# Autodesk Inventor assembly: GFBL85050-250-SET
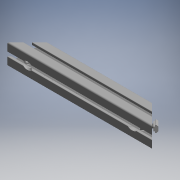
[picture p0: Inventor's stored thumbnail of the model, 180x180]
Saved by Autodesk Inventor 2017.3 (Build 213256000, 256)
## iProperties
Category: PARTsolutions
Company: MISUMI
Part Number: GFBL85050-250-SET
Catalog Web Link: www.cadenas.de
Description: GFBL8-4545,GFBL8-4590,GFBL8-5050,GFBL8-50100-Brackets for Reinforcement - HFS8-45 Series-
Vendor: MISUMI
Document SubType Name: Assembly
Designer: partserver
Manufacturer: MISUMI
Mass: 496.59 g
Surface Area: 1307.48 cm^2
Volume: 496.59 cm^3
Density: 1 g/cm^3
Title: GFBL85050-250-SET
Author: Cadenas PARTsolutions
Comments: Brackets for Reinforcement - HFS8-45 Series-
PSOL_IDENT_0: {$CADENAS_DATA\23d-libs\misumi\metric\38_al_extrusions_blackets\8_45\gfbl8_45_asmtab.prj},233 {VTYP=
PSOL_IDENT_1: 3D},{STYP=ASSTAB},{NB=GFBL85050-250-SET},{LINA=GFBL85050-250-SET},{NN=GFBL8-4545,GFBL8-4590,GFBL8-50
PSOL_IDENT_2: 50,GFBL8-50100},{DATE=08.06.2021 08:26:11},{GEOMDATE=23.05.2017 05:01:27},{VERSION=},{LINEID=30},{WB
PSOL_IDENT_3: VAR=L,ALT1},{WBNUMERIC=L}  {NB=GFBL85050-250-SET},{LINA=GFBL85050-250-SET},{KT=DUMMY},{PN=GFBL85050-
PSOL_IDENT_4: 250-SET},{TYPE=GFBL8},{NO=5050},{L=250},{ALT1=-SET},{PPATH=gfbl8_45/gfbl8_45_asmtpl.prj}
NB: GFBL85050-250-SET
NN: GFBL8-4545,GFBL8-4590,GFBL8-5050,GFBL8-50100
NT: Brackets for Reinforcement - HFS8-45 Series-
NBSYN: $PN.
LINA: GFBL85050-250-SET
CATALOG: Misumi
PN: GFBL85050-250-SET
TYPE: GFBL8
NO: 5050
L: 250
ALT1: SET Applicable Screws and Nuts Set
SUPPLIER: MISUMI
ARTICLENO: GFBL85050-250-SET
BOMINFO: GFBL85050-250-SET
CREATOR: CADENAS GmbH
## Documents named in this file (6)
- e:\temp\worker_65\temp\exporttempdir_10092_110_zDKcX\format_0\GFBL85050-250-SET.iam
- e:\temp\worker_65\temp\exporttempdir_10092_110_zDKcX\format_0\GFBL85050-250-SET_b.ipt
- e:\temp\worker_65\temp\exporttempdir_10092_110_zDKcX\format_0\HCBST8-24_Screw.ipt
- e:\temp\worker_65\temp\exporttempdir_10092_110_zDKcX\format_0\HCBST8_w1.ipt
- e:\temp\worker_65\temp\exporttempdir_10092_110_zDKcX\format_0\HCBST8washer2.ipt
- e:\temp\worker_65\temp\exporttempdir_10092_110_zDKcX\format_0\HNTT8-8.ipt
## Components (9 placed, 5 different names)
1. GFBL85050-250-SET_b:1 — to_bolt21_XY@1 <-> screw_to_body_XY@2, to_bolt21_Z@1 <-> screw_to_body_Z@2, to_bolt21_YZ@1 <-> screw_to_body_YZ@2, to_bolt22_XY@1 <-> screw_to_body_XY@5, to_bolt22_Z@1 <-> screw_to_body_Z@5, to_bolt22_YZ@1 <-> screw_to_body_YZ@5, to_nut21_XY@1 <-> to_bolt_XY@8, to_nut21_Z@1 <-> to_bolt_Z@8, to_nut21_YZ@1 <-> to_bolt_YZ@8, to_nut22_XY@1 <-> to_bolt_XY@9, to_nut22_Z@1 <-> to_bolt_Z@9, to_nut22_YZ@1 <-> to_bolt_YZ@9
2. HCBST8-24_Screw:1 — to_bolt21_XY@1 <-> screw_to_body_XY@2, to_bolt21_Z@1 <-> screw_to_body_Z@2, to_bolt21_YZ@1 <-> screw_to_body_YZ@2, bolt_to_spring_washer_XY@2 <-> spring_washer_to_bolt_XY@3, bolt_to_spring_washer_Z@2 <-> spring_washer_to_bolt_Z@3, bolt_to_spring_washer_YZ@2 <-> spring_washer_to_bolt_YZ@3, bolt_to_plane_washer_XY@2 <-> washer_to_bolt_XY@4, bolt_to_plane_washer_Z@2 <-> washer_to_bolt_Z@4, bolt_to_plane_washer_YZ@2 <-> washer_to_bolt_YZ@4
3. HCBST8_w1:1 — bolt_to_spring_washer_XY@2 <-> spring_washer_to_bolt_XY@3, bolt_to_spring_washer_Z@2 <-> spring_washer_to_bolt_Z@3, bolt_to_spring_washer_YZ@2 <-> spring_washer_to_bolt_YZ@3
4. HCBST8washer2:1 — bolt_to_plane_washer_XY@2 <-> washer_to_bolt_XY@4, bolt_to_plane_washer_Z@2 <-> washer_to_bolt_Z@4, bolt_to_plane_washer_YZ@2 <-> washer_to_bolt_YZ@4
5. HCBST8-24_Screw:2 — to_bolt22_XY@1 <-> screw_to_body_XY@5, to_bolt22_Z@1 <-> screw_to_body_Z@5, to_bolt22_YZ@1 <-> screw_to_body_YZ@5, bolt_to_spring_washer_XY@5 <-> spring_washer_to_bolt_XY@6, bolt_to_spring_washer_Z@5 <-> spring_washer_to_bolt_Z@6, bolt_to_spring_washer_YZ@5 <-> spring_washer_to_bolt_YZ@6, bolt_to_plane_washer_XY@5 <-> washer_to_bolt_XY@7, bolt_to_plane_washer_Z@5 <-> washer_to_bolt_Z@7, bolt_to_plane_washer_YZ@5 <-> washer_to_bolt_YZ@7
6. HCBST8_w1:2 — bolt_to_spring_washer_XY@5 <-> spring_washer_to_bolt_XY@6, bolt_to_spring_washer_Z@5 <-> spring_washer_to_bolt_Z@6, bolt_to_spring_washer_YZ@5 <-> spring_washer_to_bolt_YZ@6
7. HCBST8washer2:2 — bolt_to_plane_washer_XY@5 <-> washer_to_bolt_XY@7, bolt_to_plane_washer_Z@5 <-> washer_to_bolt_Z@7, bolt_to_plane_washer_YZ@5 <-> washer_to_bolt_YZ@7
8. HNTT8-8:1 — to_nut21_XY@1 <-> to_bolt_XY@8, to_nut21_Z@1 <-> to_bolt_Z@8, to_nut21_YZ@1 <-> to_bolt_YZ@8
9. HNTT8-8:2 — to_nut22_XY@1 <-> to_bolt_XY@9, to_nut22_Z@1 <-> to_bolt_Z@9, to_nut22_YZ@1 <-> to_bolt_YZ@9
## Relationships (24: Mate 14, Angle 8, Flush 2)
- to_bolt21_XY@1 <-> screw_to_body_XY@2 [Mate] (4.2 mm): GFBL85050-250-SET_b:1 ↔ HCBST8-24_Screw:1
- to_bolt21_Z@1 <-> screw_to_body_Z@2 [Mate]: GFBL85050-250-SET_b:1 ↔ HCBST8-24_Screw:1
- to_bolt21_YZ@1 <-> screw_to_body_YZ@2 [Angle] (0 deg): GFBL85050-250-SET_b:1 ↔ HCBST8-24_Screw:1
- bolt_to_spring_washer_XY@2 <-> spring_washer_to_bolt_XY@3 [Mate] (-2.8 mm): HCBST8-24_Screw:1 ↔ HCBST8_w1:1
- bolt_to_spring_washer_Z@2 <-> spring_washer_to_bolt_Z@3 [Mate]: HCBST8-24_Screw:1 ↔ HCBST8_w1:1
- bolt_to_spring_washer_YZ@2 <-> spring_washer_to_bolt_YZ@3 [Angle] (0 deg): HCBST8-24_Screw:1 ↔ HCBST8_w1:1
- bolt_to_plane_washer_XY@2 <-> washer_to_bolt_XY@4 [Mate] (-3.5 mm): HCBST8-24_Screw:1 ↔ HCBST8washer2:1
- bolt_to_plane_washer_Z@2 <-> washer_to_bolt_Z@4 [Mate]: HCBST8-24_Screw:1 ↔ HCBST8washer2:1
- bolt_to_plane_washer_YZ@2 <-> washer_to_bolt_YZ@4 [Angle] (0 deg): HCBST8-24_Screw:1 ↔ HCBST8washer2:1
- to_bolt22_XY@1 <-> screw_to_body_XY@5 [Mate] (4.2 mm): GFBL85050-250-SET_b:1 ↔ HCBST8-24_Screw:2
- to_bolt22_Z@1 <-> screw_to_body_Z@5 [Mate]: GFBL85050-250-SET_b:1 ↔ HCBST8-24_Screw:2
- to_bolt22_YZ@1 <-> screw_to_body_YZ@5 [Angle] (0 deg): GFBL85050-250-SET_b:1 ↔ HCBST8-24_Screw:2
- bolt_to_spring_washer_XY@5 <-> spring_washer_to_bolt_XY@6 [Mate] (-2.8 mm): HCBST8-24_Screw:2 ↔ HCBST8_w1:2
- bolt_to_spring_washer_Z@5 <-> spring_washer_to_bolt_Z@6 [Mate]: HCBST8-24_Screw:2 ↔ HCBST8_w1:2
- bolt_to_spring_washer_YZ@5 <-> spring_washer_to_bolt_YZ@6 [Angle] (0 deg): HCBST8-24_Screw:2 ↔ HCBST8_w1:2
- bolt_to_plane_washer_XY@5 <-> washer_to_bolt_XY@7 [Mate] (-3.5 mm): HCBST8-24_Screw:2 ↔ HCBST8washer2:2
- bolt_to_plane_washer_Z@5 <-> washer_to_bolt_Z@7 [Mate]: HCBST8-24_Screw:2 ↔ HCBST8washer2:2
- bolt_to_plane_washer_YZ@5 <-> washer_to_bolt_YZ@7 [Angle] (0 deg): HCBST8-24_Screw:2 ↔ HCBST8washer2:2
- to_nut21_XY@1 <-> to_bolt_XY@8 [Flush] (-19.8 mm): GFBL85050-250-SET_b:1 ↔ HNTT8-8:1
- to_nut21_Z@1 <-> to_bolt_Z@8 [Mate]: GFBL85050-250-SET_b:1 ↔ HNTT8-8:1
- to_nut21_YZ@1 <-> to_bolt_YZ@8 [Angle] (90 deg): GFBL85050-250-SET_b:1 ↔ HNTT8-8:1
- to_nut22_XY@1 <-> to_bolt_XY@9 [Flush] (-19.8 mm): GFBL85050-250-SET_b:1 ↔ HNTT8-8:2
- to_nut22_Z@1 <-> to_bolt_Z@9 [Mate]: GFBL85050-250-SET_b:1 ↔ HNTT8-8:2
- to_nut22_YZ@1 <-> to_bolt_YZ@9 [Angle] (90 deg): GFBL85050-250-SET_b:1 ↔ HNTT8-8:2
